# Autodesk Inventor assembly: Montagem dianteria completa
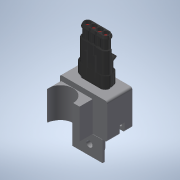
[picture p0: Inventor's stored thumbnail of the model, 180x180]
Saved by Autodesk Inventor 2021 (Build 250183000, 183)
## iProperties
Created: 2021-06-28
Part Number: Montagem dianteria completa
Material: Genérico
Document SubType Name: Assembly
Designer: SOU O MELHOR
Author: SOU O MELHOR
## Documents named in this file (5)
- G:\Meu Drive\Projetos\Projeto 2020 2021\Eletrônica 2020-2021\Projeção mecânica\Nova fixação do acelerometro 2\Montagem dianteria completa.iam
- G:\Meu Drive\Projetos\Projeto 2020 2021\Eletrônica 2020-2021\Projeção mecânica\Nova fixação do acelerometro 2\Caixa dianteira.ipt
- G:\Meu Drive\Projetos\Projeto 2020 2021\Eletrônica 2020-2021\Projeção mecânica\Nova fixação do acelerometro 2\Fixador acelerometro dianteiro.ipt
- G:\Meu Drive\Projetos\Projeto 2020 2021\Eletrônica 2020-2021\Projeção mecânica\Nova fixação do acelerometro 2\MPU6050.ipt
- G:\Meu Drive\Projetos\Projeto 2020 2021\Eletrônica 2020-2021\Projeção mecânica\Nova fixação do acelerometro 2\AMP 4 position.ipt
## Components (4 placed, 4 different names)
1. Caixa dianteira:1 — Coincidência:1, Rotativa:1, Coincidente:2, Coincidente:3, Coincidente:4
2. Fixador acelerometro dianteiro:1 — Coincidência:1, Coincidente:4
3. MPU6050:1 — Rotativa:1
4. AMP 4 position:1 — Coincidente:2, Coincidente:3
## Relationships (5: Mate 4, RevoluteJoint 1)
- Coincidência:1 [Mate]: Caixa dianteira:1 ↔ Fixador acelerometro dianteiro:1
- Rotativa:1 [RevoluteJoint] (-0.5 mm): Caixa dianteira:1 ↔ MPU6050:1
- Coincidente:2 [Mate]: Caixa dianteira:1 ↔ AMP 4 position:1
- Coincidente:3 [Mate]: Caixa dianteira:1 ↔ AMP 4 position:1
- Coincidente:4 [Mate]: Caixa dianteira:1 ↔ Fixador acelerometro dianteiro:1
